# Autodesk Inventor assembly: Montagem1
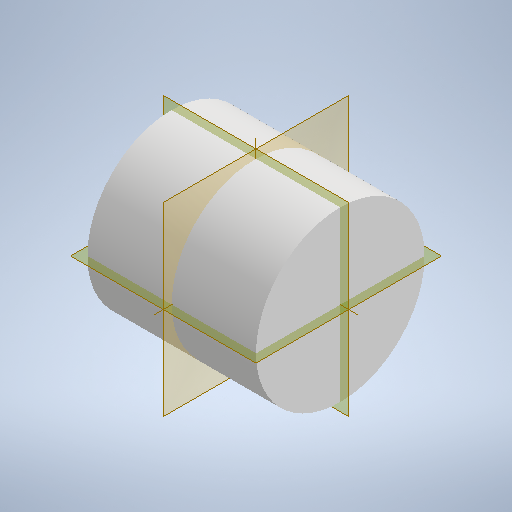
[picture p0: Inventor's stored thumbnail of the model, 512x512]
Saved by Autodesk Inventor 2026 (Build 300175000, 175)
## iProperties
Created: 2025-03-25
Part Number: Montagem1
Document SubType Name: Assembly
Designer: Carlos Dias
Author: Carlos Dias
## Documents named in this file (2)
- C:\Users\Carlos Dias\Documents\Formação-TEARCI\UFCDs\5134 - Robótica _ Fundamentos\Material De Apoio\Assembly\Montagem1.iam
- C:\Users\Carlos Dias\Documents\Formação-TEARCI\UFCDs\5134 - Robótica _ Fundamentos\Material De Apoio\Assembly\peca_011_001.ipt
## Components (1 placed, 1 different names)
1. peca_011_001:1 — Mate:1, Mate:2, Flush:1
## Relationships (3: Mate 2, Flush 1)
- Mate:1: peca_011_001:1
- Mate:2: peca_011_001:1
- Flush:1: peca_011_001:1
